# Autodesk Inventor assembly: easy_door
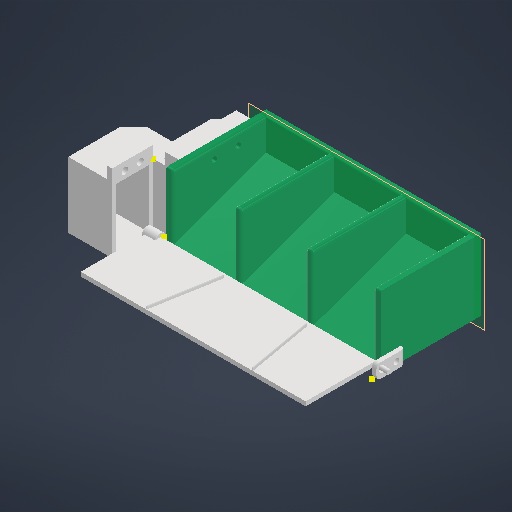
[picture p0: Inventor's stored thumbnail of the model, 512x512]
Saved by Autodesk Inventor 2026.1 (Build 301233000, 233)
## iProperties
Created: 2026-03-14
Part Number: easy_door
Document SubType Name: Assembly
Designer: ba2032
Author: ba2032
## Documents named in this file (6)
- H:\CAD Project\robot project\Easy Door\container-door-assembly-group2.iam
- H:\CAD Project\robot project\Easy Door\container-door-group2.ipt
- H:\CAD Project\robot project\Easy Door\holder 1.ipt
- H:\CAD Project\robot project\Easy Door\rubbish-container-group2.ipt
- H:\CAD Project\robot project\Easy Door\container-door-holder-group2.ipt
- H:\CAD Project\robot project\Easy Door\container-servo-holder-group2.ipt
## Components (5 placed, 5 different names)
1. holder 1:1
2. rubbish-container-group2:1 — Rigid:1, Rigid:2
3. container-door-holder-group2:1 — Rigid:1, Rotational:1
4. container-door-group2:1 — Rotational:1
5. container-servo-holder-group2:1 — Rigid:2
## Relationships (3: WeldJoint 2, RevoluteJoint 1)
- Rigid:1 [WeldJoint]: rubbish-container-group2:1 ↔ container-door-holder-group2:1
- Rotational:1 [RevoluteJoint] (-6 mm): container-door-holder-group2:1 ↔ container-door-group2:1
- Rigid:2 [WeldJoint]: rubbish-container-group2:1 ↔ container-servo-holder-group2:1
